# Autodesk Inventor assembly: bett_V2_bein
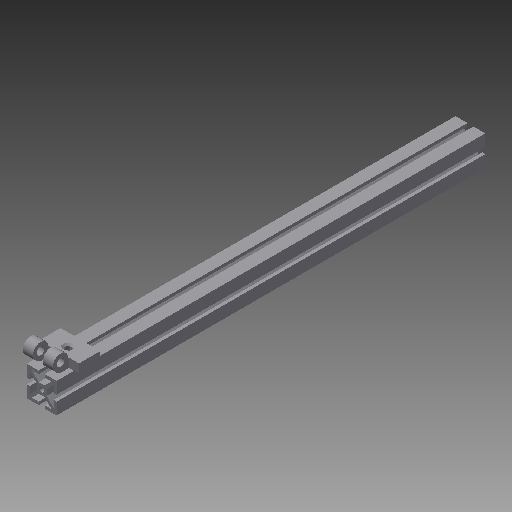
[picture p0: Inventor's stored thumbnail of the model, 512x512]
Saved by Autodesk Inventor 2018 (Build 220112000, 112)
## iProperties
Created: 2020-04-19
Part Number: bett_V2_bein
Material: Generisch
Document SubType Name: Assembly
Designer: wepet
Author: wepet
## Documents named in this file (3)
- C:\Users\wepet\Downloads\anhaenger\current\details\bett\bett_V2\bett_V2_teil4_bein.iam
- C:\Users\wepet\Downloads\anhaenger\current\details\bett\details\item_30x30_43cm.ipt
- C:\Users\wepet\Downloads\anhaenger\current\details\bett\details\item_scharnier_1_teil.ipt
## Components (2 placed, 2 different names)
1. item_30x30_43cm:1 — Passend:1, Fluchtend:1, Passend:2
2. item_scharnier_1_teil:1 — Passend:1, Fluchtend:1, Passend:2
## Relationships (3: Mate 2, Flush 1)
- Passend:1 [Mate]: item_30x30_43cm:1 ↔ item_scharnier_1_teil:1
- Fluchtend:1 [Flush] (-0.5 mm): item_30x30_43cm:1 ↔ item_scharnier_1_teil:1
- Passend:2 [Mate] (-3.9 mm): item_30x30_43cm:1 ↔ item_scharnier_1_teil:1
